# Autodesk Inventor assembly: MAIN
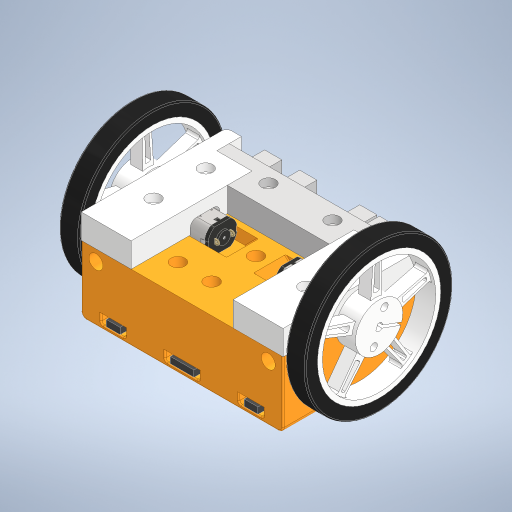
[picture p0: Inventor's stored thumbnail of the model, 512x512]
Saved by Autodesk Inventor 2023 (Build 270158000, 158)
## iProperties
Created: 2024-04-25
Part Number: MAIN
Document SubType Name: Assembly
Designer: Kamil
Author: Kamil
## Documents named in this file (13)
- C:\Users\Kamil\Documents\PROJEKT ZESPOLOWY\mechanics\MAIN.iam
- C:\Users\Kamil\Documents\PROJEKT ZESPOLOWY\mechanics\PololuWheel 60x8mm.ipt
- C:\Users\Kamil\Documents\PROJEKT ZESPOLOWY\mechanics\N20 DC MOTOR.ipt
- C:\Users\Kamil\Documents\PROJEKT ZESPOLOWY\mechanics\podst.ipt
- C:\Users\Kamil\Documents\PROJEKT ZESPOLOWY\mechanics\Li_Pol 800mAh.ipt
- C:\Users\Kamil\Documents\PROJEKT ZESPOLOWY\mechanics\pokrywka_baterii.ipt
- C:\Users\Kamil\Documents\PROJEKT ZESPOLOWY\mechanics\prod.ipt
- C:\Users\Kamil\Documents\PROJEKT ZESPOLOWY\mechanics\PCB_MAIN.ipt
- C:\Users\Kamil\Documents\PROJEKT ZESPOLOWY\mechanics\N20_Bracket_Extended_Pololu.ipt
- C:\Users\Kamil\Documents\PROJEKT ZESPOLOWY\mechanics\N20_Bracket_Extended_Pololu_MIR.ipt
- C:\Users\Kamil\Documents\PROJEKT ZESPOLOWY\mechanics\tyl.ipt
- C:\Users\Kamil\Documents\PROJEKT ZESPOLOWY\mechanics\literka.ipt
- C:\Users\Kamil\Documents\PROJEKT ZESPOLOWY\mechanics\podstawka_na_pcb.ipt
## Components (17 placed, 12 different names)
1. PololuWheel 60x8mm:1 — Zestawiające:1, Kątowe:1, Zestawiające:2, Zestawiające:5, Zestawiające:6, Równoległe:2
2. N20 DC MOTOR:1 — Zestawiające:1, Kątowe:1, Zestawiające:2, Równoległe:1, Zestawiające:9, Zestawiające:18, Zestawiające:19
3. PololuWheel 60x8mm:2 — Zestawiające:5, Zestawiające:6, Zestawiające:10, Równoległe:7
4. N20 DC MOTOR:2 — Równoległe:1, Zestawiające:7
5. podst:1 — Zestawiające:9, Zestawiające:10, Zestawiające:11, Zestawiające:12, Zestawiające:13, Równoległe:6, Zestawiające:14, Zestawiające:15, Zestawiające:16, Równoległe:8, Zestawiające:20, Równoległe:15
6. Li_Pol 800mAh:1 — Zestawiające:11, Zestawiające:12, Zestawiające:13
7. pokrywka_baterii:1 — Równoległe:6, Zestawiające:14, Zestawiające:15
8. prod:1 — Zestawiające:16, Równoległe:7, Równoległe:8
9. PCB_MAIN:1 — Zestawiające:28
10. N20_Bracket_Extended_Pololu:1 — Zestawiające:18, Zestawiające:19, Zestawiające:21, Zestawiające:23, Zestawiające:27
11. N20_Bracket_Extended_Pololu_MIR:1 — Równoległe:16
12. tyl:1 — Zestawiające:20, Zestawiające:21, Zestawiające:22, Równoległe:11, Zestawiające:23, Zestawiające:24, Zestawiające:25, Zestawiające:26, Równoległe:12, Równoległe:13, Równoległe:14
13. literka:1 — Zestawiające:22, Równoległe:11
14. literka:2 — Zestawiające:24, Równoległe:14
15. literka:3 — Zestawiające:25, Równoległe:13
16. literka:4 — Zestawiające:26, Równoległe:12
17. podstawka_na_pcb:1 — Zestawiające:27, Równoległe:15, Równoległe:16, Zestawiające:28
## Relationships (39: Mate 26, Flush 11, Angle 2)
- Zestawiające:1 [Mate]: PololuWheel 60x8mm:1 ↔ N20 DC MOTOR:1
- Kątowe:1 [Angle] (180 deg): PololuWheel 60x8mm:1 ↔ N20 DC MOTOR:1
- Zestawiające:2 [Mate]: PololuWheel 60x8mm:1 ↔ N20 DC MOTOR:1
- [Mate]: PololuWheel 60x8mm:2 ↔ N20 DC MOTOR:2
- [Angle] (180 deg): PololuWheel 60x8mm:2 ↔ N20 DC MOTOR:2
- [Mate]: PololuWheel 60x8mm:2 ↔ N20 DC MOTOR:2
- Zestawiające:5 [Mate]: PololuWheel 60x8mm:1 ↔ PololuWheel 60x8mm:2
- Równoległe:1 [Flush]: N20 DC MOTOR:1 ↔ N20 DC MOTOR:2
- Zestawiające:6 [Mate] (-100 mm): PololuWheel 60x8mm:1 ↔ PololuWheel 60x8mm:2
- Zestawiające:7 [Mate]: N20 DC MOTOR:2
- Równoległe:2 [Flush]: PololuWheel 60x8mm:1
- Zestawiające:9 [Mate]: N20 DC MOTOR:1 ↔ podst:1
- Zestawiające:10 [Mate] (1 mm): PololuWheel 60x8mm:2 ↔ podst:1
- Zestawiające:11 [Mate]: podst:1 ↔ Li_Pol 800mAh:1
- Zestawiające:12 [Mate] (0.5 mm): podst:1 ↔ Li_Pol 800mAh:1
- Zestawiające:13 [Mate] (6 mm): podst:1 ↔ Li_Pol 800mAh:1
- Równoległe:6 [Flush]: podst:1 ↔ pokrywka_baterii:1
- Zestawiające:14 [Mate]: podst:1 ↔ pokrywka_baterii:1
- Zestawiające:15 [Mate]: podst:1 ↔ pokrywka_baterii:1
- Zestawiające:16 [Mate]: podst:1 ↔ prod:1
- Równoległe:7 [Flush]: PololuWheel 60x8mm:2 ↔ prod:1
- Równoległe:8 [Flush]: podst:1 ↔ prod:1
- Zestawiające:18 [Mate]: N20 DC MOTOR:1 ↔ N20_Bracket_Extended_Pololu:1
- Zestawiające:19 [Mate]: N20 DC MOTOR:1 ↔ N20_Bracket_Extended_Pololu:1
- Zestawiające:20 [Mate]: podst:1 ↔ tyl:1
- Zestawiające:21 [Mate]: N20_Bracket_Extended_Pololu:1 ↔ tyl:1
- Zestawiające:22 [Mate]: tyl:1 ↔ literka:1
- Równoległe:11 [Flush]: tyl:1 ↔ literka:1
- Zestawiające:23 [Mate]: N20_Bracket_Extended_Pololu:1 ↔ tyl:1
- Zestawiające:24 [Mate]: tyl:1 ↔ literka:2
- Zestawiające:25 [Mate]: tyl:1 ↔ literka:3
- Zestawiające:26 [Mate]: tyl:1 ↔ literka:4
- Równoległe:12 [Flush]: tyl:1 ↔ literka:4
- Równoległe:13 [Flush]: tyl:1 ↔ literka:3
- Równoległe:14 [Flush]: tyl:1 ↔ literka:2
- Zestawiające:27 [Mate]: N20_Bracket_Extended_Pololu:1 ↔ podstawka_na_pcb:1
- Równoległe:15 [Flush]: podst:1 ↔ podstawka_na_pcb:1
- Równoległe:16 [Flush]: N20_Bracket_Extended_Pololu_MIR:1 ↔ podstawka_na_pcb:1
- Zestawiające:28 [Mate]: PCB_MAIN:1 ↔ podstawka_na_pcb:1
## Named parameters: d3_d2 = 0 mm, d4_d0 = 0 mm, d5_d1 = 180 deg
